# Autodesk Inventor assembly: Z
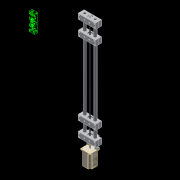
[picture p0: Inventor's stored thumbnail of the model, 180x180]
Saved by Autodesk Inventor 2016 (Build 200138000, 138)
## iProperties
Created: 2017-07-13
Part Number: Z
Document SubType Name: Assembly
Designer: ludwi
Author: ludwi
## Documents named in this file (8)
- H:\MARQ\3D\AXIS_DEV_EDT_V3\Y.iam
- H:\MARQ\3D\AXIS_DEV_EDT_V3\AXB.ipt
- C:\Users\ludwi\OneDrive\Documentos\Inventor\Content Center Files\R2016\en-US\DIN BEARING(1)\DIN 625 SKF - SKF 626.ipt
- C:\Users\ludwi\OneDrive\Documentos\Inventor\Content Center Files\R2016\en-US\DIN 935\DIN 935 T1 - M6 x 1 x 10.ipt
- H:\MARQ\3D\AXIS_DEV_EDT_V3\NEMA23.ipt
- H:\MARQ\3D\AXIS_DEV_EDT_V3\MSUP.ipt
- H:\MARQ\3D\AXIS_DEV_EDT_V3\TuboEstructura.ipt
- H:\MARQ\3D\AXIS_DEV_EDT_V3\M6SM.ipt
## Components (17 placed, 7 different names)
1. AXB:1 — Insert:9, Insert:19, Mate:14
2. AXB:2 — Insert:16, Insert:17
3. AXB:3 — Insert:10
4. AXB:4 — Insert:18, Mate:14
5. DIN 625 SKF SKF 626:1 — Insert:9, Mate:6
6. DIN 625 SKF SKF 626:2 — Insert:10, Mate:4
7. DIN 935 M6:1 — Mate:4
8. DIN 935 M6:2 — Mate:6
9. NEMA23:1 — Insert:13, Insert:14, Insert:20
10. MSUP:2 — Insert:13, Insert:14
11. TuboEstructura:1 — Insert:16, Insert:18, Mate:20, Mate:22
12. TuboEstructura:2 — Insert:17, Insert:19, Mate:19, Mate:21
13. M6SM:1 — Insert:20
14. AXB:5 — Mate:16, Flush:1, Flush:2, Mate:19, Mate:20
15. AXB:6 — Mate:16, Flush:1, Flush:2
16. AXB:7
17. AXB:8 — Mate:21, Mate:22
## Relationships (24: Mate 11, Insert 9, Flush 4)
- Insert:9: AXB:1 ↔ DIN 625 SKF SKF 626:1
- Insert:10: AXB:3 ↔ DIN 625 SKF SKF 626:2
- Mate:4: DIN 625 SKF SKF 626:2 ↔ DIN 935 M6:1
- Mate:6: DIN 625 SKF SKF 626:1 ↔ DIN 935 M6:2
- Insert:13: NEMA23:1 ↔ MSUP:2
- Insert:14: NEMA23:1 ↔ MSUP:2
- Insert:16: AXB:2 ↔ TuboEstructura:1
- Insert:17: AXB:2 ↔ TuboEstructura:2
- Insert:18: AXB:4 ↔ TuboEstructura:1
- Insert:19: AXB:1 ↔ TuboEstructura:2
- Insert:20: NEMA23:1 ↔ M6SM:1
- Mate:14: AXB:1 ↔ AXB:4
- [Mate]: AXB:5 ↔ AXB:6
- Mate:16: AXB:5 ↔ AXB:6
- Flush:1: AXB:5 ↔ AXB:6
- Flush:2: AXB:5 ↔ AXB:6
- [Mate]: AXB:7 ↔ AXB:8
- [Mate]: AXB:7 ↔ AXB:8
- [Flush]: AXB:7 ↔ AXB:8
- [Flush]: AXB:7 ↔ AXB:8
- Mate:19: TuboEstructura:2 ↔ AXB:5
- Mate:20: TuboEstructura:1 ↔ AXB:5
- Mate:21: TuboEstructura:2 ↔ AXB:8
- Mate:22: TuboEstructura:1 ↔ AXB:8
## Named parameters: d48_d43 = 0 mm, d52_d49 = 0 mm, d53_d50 = 0 mm, d54_d51 = 0 mm, d55_d48_d43 = 0 mm
